# Autodesk Inventor assembly: X-Axis
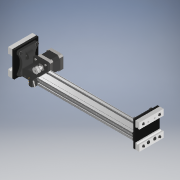
[picture p0: Inventor's stored thumbnail of the model, 180x180]
Saved by Autodesk Inventor 2020.2 (Build 242310000, 310)
## iProperties
Created: 2020-04-02
Part Number: X-Axis
Document SubType Name: Assembly
Designer: rah75
Author: rah75
## Documents named in this file (19)
- C:\Users\rah75\Documents\GitHub\LETU-Maker\CAD\Autodesk Inventor\Base_3001-5999\X-Axis\Assemblies\X-Axis.iam
- C:\Users\rah75\Documents\GitHub\LETU-Maker\CAD\Autodesk Inventor\Base_3001-5999\X-Axis\Fabricated_Parts\X-Axis_Makerslide_LM3003.ipt
- C:\Users\rah75\Documents\GitHub\LETU-Maker\CAD\Autodesk Inventor\Base_3001-5999\X-Axis\Printed_Parts\X-Axis_Carriage_Mount_L_LM3001.ipt
- C:\Users\rah75\Documents\GitHub\LETU-Maker\CAD\Autodesk Inventor\Base_3001-5999\X-Axis\Printed_Parts\X-Axis_Carriage_Mount_R_LM3002.ipt
- C:\Users\rah75\Documents\GitHub\LETU-Maker\CAD\Autodesk Inventor\Base_3001-5999\X-Axis\Fabricated_Parts\X-Axis_End_Plate_LM3004.ipt
- C:\Users\rah75\Documents\GitHub\LETU-Maker\CAD\Autodesk Inventor\Base_3001-5999\X-Axis\Printed_Parts\X-Axis_Mount_Slide_LM3005.ipt
- C:\Users\rah75\Documents\GitHub\LETU-Maker\CAD\Autodesk Inventor\Stock_Components_1001-2999\Motors\NEMA_17_LM1028.ipt
- C:\Users\rah75\Documents\GitHub\LETU-Maker\CAD\Autodesk Inventor\Stock_Components_1001-2999\Power_Transmission\GT2_pulley_LM1034.ipt
- C:\Users\rah75\Documents\GitHub\LETU-Maker\CAD\Autodesk Inventor\Stock_Components_1001-2999\Fasteners\Nuts\hex_nut_m5_LM1020.ipt
- C:\Users\rah75\Documents\GitHub\LETU-Maker\CAD\Autodesk Inventor\Stock_Components_1001-2999\Fasteners\Washers_Spacers\washer_m5_LM1002.ipt
- C:\Users\rah75\Documents\GitHub\LETU-Maker\CAD\Autodesk Inventor\Stock_Components_1001-2999\Fasteners\Screws\BHHD_m5x30_LM1004.ipt
- C:\Users\rah75\Documents\GitHub\LETU-Maker\CAD\Autodesk Inventor\Stock_Components_1001-2999\Fasteners\Screws\SHCS_m3x8_LM1008.ipt
- C:\Users\rah75\Documents\GitHub\LETU-Maker\CAD\Autodesk Inventor\Stock_Components_1001-2999\Fasteners\Screws\SHCS_m3x30_LM1012.ipt
- C:\Users\rah75\Documents\GitHub\LETU-Maker\CAD\Autodesk Inventor\Stock_Components_1001-2999\Power_Transmission\Bearings\623-SS_3x10mm_LM1029.ipt
- C:\Users\rah75\Documents\GitHub\LETU-Maker\CAD\Autodesk Inventor\Stock_Components_1001-2999\Fasteners\Screws\BHHD_m5x45_LM1005.ipt
- C:\Users\rah75\Documents\GitHub\LETU-Maker\CAD\Autodesk Inventor\Stock_Components_1001-2999\Fasteners\Screws\BHHS_m5x80_LM1039.ipt
- C:\Users\rah75\Documents\GitHub\LETU-Maker\CAD\Autodesk Inventor\Stock_Components_1001-2999\Electrical\limit_switch_LM1025.ipt
- C:\Users\rah75\Documents\GitHub\LETU-Maker\CAD\Autodesk Inventor\Stock_Components_1001-2999\Fasteners\Screws\BHHD_m2x10_LM1040.ipt
- C:\Users\rah75\Documents\GitHub\LETU-Maker\CAD\Autodesk Inventor\Stock_Components_1001-2999\Springs\spring_7_5x10mm_LM1036.ipt
## Components (48 placed, 18 different names)
1. X-Axis_Makerslide_LM3003:1 — Insert:1, Mate:1, Insert:2, Mate:2
2. X-Axis_Carriage_Mount_L_LM3001:1 — Insert:2, Mate:2, Insert:4, Mate:4, Insert:8, Mate:10, Insert:25, Insert:26, Insert:28, Insert:29, Insert:30, Insert:31, Insert:32, Insert:40, Mate:11, Insert:43, Mate:14
3. X-Axis_Carriage_Mount_R_LM3002:1 — Insert:1, Mate:1, Insert:3, Mate:3, Mate:7, Insert:18, Insert:20, Insert:22, Insert:27, Insert:33, Insert:35, Mate:12, Mate:13, Angle:1, Mate:16, Mate:17
4. X-Axis_End_Plate_LM3004:1 — Insert:3, Mate:3, Insert:5, Mate:5, Mate:6
5. X-Axis_End_Plate_LM3004:2 — Insert:4, Mate:4, Insert:6, Mate:8, Insert:7, Mate:9
6. X-Axis_Mount_Slide_LM3005:1 — Insert:6, Mate:8, Insert:12, Insert:13, Insert:38, Insert:39
7. X-Axis_Mount_Slide_LM3005:2 — Insert:7, Mate:9, Insert:10, Insert:11
8. X-Axis_Mount_Slide_LM3005:3 — Flush:1, Mate:6, Mate:7, Insert:14, Insert:17
9. X-Axis_Mount_Slide_LM3005:4 — Insert:5, Mate:5, Flush:1, Insert:15, Insert:16, Insert:36, Insert:37
10. NEMA_17_LM1028:1 — Insert:8, Mate:10, Insert:9
11. GT2_pulley_LM1034:1 — Insert:9
12. hex_nut_m5_LM1020:1 — Insert:16
13. hex_nut_m5_LM1020:2 — Insert:12
14. hex_nut_m5_LM1020:3 — Insert:11
15. hex_nut_m5_LM1020:4 — Insert:10
16. hex_nut_m5_LM1020:5 — Insert:15
17. hex_nut_m5_LM1020:6 — Insert:14
18. hex_nut_m5_LM1020:7 — Insert:13
19. hex_nut_m5_LM1020:8 — Insert:17
20. washer_m5_LM1002:1 — Insert:24, Insert:26
21. washer_m5_LM1002:2 — Insert:23, Insert:25
22. washer_m5_LM1002:3 — Insert:19, Insert:20
23. washer_m5_LM1002:4 — Insert:21, Insert:22
24. BHHD_m5x30_LM1004:1 — Insert:23
25. BHHD_m5x30_LM1004:2 — Insert:24
26. BHHD_m5x30_LM1004:3 — Insert:19
27. BHHD_m5x30_LM1004:4 — Insert:21
28. BHHD_m5x30_LM1004:5 — Insert:18
29. BHHD_m5x30_LM1004:6 — Insert:28
30. BHHD_m5x30_LM1004:7 — Insert:27
31. BHHD_m5x30_LM1004:8 — Insert:29
32. SHCS_m3x8_LM1008:1 — Insert:30
33. SHCS_m3x8_LM1008:2 — Insert:31
34. SHCS_m3x8_LM1008:3 — Insert:32
35. SHCS_m3x30_LM1012:1 — Insert:33
36. 623-SS_3x10mm_LM1029:1 — Insert:34
37. 623-SS_3x10mm_LM1029:2 — Insert:34, Insert:35
38. BHHD_m5x45_LM1005:1 — Insert:36
39. BHHD_m5x45_LM1005:2 — Insert:37
40. BHHS_m5x80_LM1039:1 — Insert:38
41. BHHS_m5x80_LM1039:2 — Insert:39
42. limit_switch_LM1025:1 — Insert:40, Mate:11, Insert:41, Insert:42
43. BHHD_m2x10_LM1040:1 — Insert:41
44. BHHD_m2x10_LM1040:2 — Insert:42
45. hex_nut_m5_LM1020:9 — Mate:12, Mate:13, Angle:1
46. hex_nut_m5_LM1020:10 — Insert:43, Mate:15
47. spring_7_5x10mm_LM1036:1 — Mate:14, Mate:15
48. spring_7_5x10mm_LM1036:2 — Mate:16, Mate:17
## Relationships (62: Insert 43, Mate 17, Flush 1, Angle 1)
- Insert:1: X-Axis_Makerslide_LM3003:1 ↔ X-Axis_Carriage_Mount_R_LM3002:1
- Mate:1: X-Axis_Makerslide_LM3003:1 ↔ X-Axis_Carriage_Mount_R_LM3002:1
- Insert:2: X-Axis_Makerslide_LM3003:1 ↔ X-Axis_Carriage_Mount_L_LM3001:1
- Mate:2: X-Axis_Makerslide_LM3003:1 ↔ X-Axis_Carriage_Mount_L_LM3001:1
- Insert:3: X-Axis_Carriage_Mount_R_LM3002:1 ↔ X-Axis_End_Plate_LM3004:1
- Mate:3: X-Axis_Carriage_Mount_R_LM3002:1 ↔ X-Axis_End_Plate_LM3004:1
- Insert:4: X-Axis_Carriage_Mount_L_LM3001:1 ↔ X-Axis_End_Plate_LM3004:2
- Mate:4: X-Axis_Carriage_Mount_L_LM3001:1 ↔ X-Axis_End_Plate_LM3004:2
- Insert:5: X-Axis_End_Plate_LM3004:1 ↔ X-Axis_Mount_Slide_LM3005:4
- Mate:5: X-Axis_End_Plate_LM3004:1 ↔ X-Axis_Mount_Slide_LM3005:4
- Flush:1: X-Axis_Mount_Slide_LM3005:3 ↔ X-Axis_Mount_Slide_LM3005:4
- Mate:6: X-Axis_End_Plate_LM3004:1 ↔ X-Axis_Mount_Slide_LM3005:3
- Mate:7: X-Axis_Carriage_Mount_R_LM3002:1 ↔ X-Axis_Mount_Slide_LM3005:3
- Insert:6: X-Axis_End_Plate_LM3004:2 ↔ X-Axis_Mount_Slide_LM3005:1
- Mate:8: X-Axis_End_Plate_LM3004:2 ↔ X-Axis_Mount_Slide_LM3005:1
- Insert:7: X-Axis_End_Plate_LM3004:2 ↔ X-Axis_Mount_Slide_LM3005:2
- Mate:9: X-Axis_End_Plate_LM3004:2 ↔ X-Axis_Mount_Slide_LM3005:2
- Insert:8: X-Axis_Carriage_Mount_L_LM3001:1 ↔ NEMA_17_LM1028:1
- Mate:10: X-Axis_Carriage_Mount_L_LM3001:1 ↔ NEMA_17_LM1028:1
- Insert:9 (5 mm): NEMA_17_LM1028:1 ↔ GT2_pulley_LM1034:1
- Insert:10: X-Axis_Mount_Slide_LM3005:2 ↔ hex_nut_m5_LM1020:4
- Insert:11: X-Axis_Mount_Slide_LM3005:2 ↔ hex_nut_m5_LM1020:3
- Insert:12: X-Axis_Mount_Slide_LM3005:1 ↔ hex_nut_m5_LM1020:2
- Insert:13: X-Axis_Mount_Slide_LM3005:1 ↔ hex_nut_m5_LM1020:7
- Insert:14: X-Axis_Mount_Slide_LM3005:3 ↔ hex_nut_m5_LM1020:6
- Insert:15: X-Axis_Mount_Slide_LM3005:4 ↔ hex_nut_m5_LM1020:5
- Insert:16: X-Axis_Mount_Slide_LM3005:4 ↔ hex_nut_m5_LM1020:1
- Insert:17: X-Axis_Mount_Slide_LM3005:3 ↔ hex_nut_m5_LM1020:8
- Insert:18: X-Axis_Carriage_Mount_R_LM3002:1 ↔ BHHD_m5x30_LM1004:5
- Insert:19: washer_m5_LM1002:3 ↔ BHHD_m5x30_LM1004:3
- Insert:20: X-Axis_Carriage_Mount_R_LM3002:1 ↔ washer_m5_LM1002:3
- Insert:21: washer_m5_LM1002:4 ↔ BHHD_m5x30_LM1004:4
- Insert:22: X-Axis_Carriage_Mount_R_LM3002:1 ↔ washer_m5_LM1002:4
- Insert:23: washer_m5_LM1002:2 ↔ BHHD_m5x30_LM1004:1
- Insert:24: washer_m5_LM1002:1 ↔ BHHD_m5x30_LM1004:2
- Insert:25: X-Axis_Carriage_Mount_L_LM3001:1 ↔ washer_m5_LM1002:2
- Insert:26: X-Axis_Carriage_Mount_L_LM3001:1 ↔ washer_m5_LM1002:1
- Insert:27: X-Axis_Carriage_Mount_R_LM3002:1 ↔ BHHD_m5x30_LM1004:7
- Insert:28: X-Axis_Carriage_Mount_L_LM3001:1 ↔ BHHD_m5x30_LM1004:6
- Insert:29: X-Axis_Carriage_Mount_L_LM3001:1 ↔ BHHD_m5x30_LM1004:8
- Insert:30: X-Axis_Carriage_Mount_L_LM3001:1 ↔ SHCS_m3x8_LM1008:1
- Insert:31: X-Axis_Carriage_Mount_L_LM3001:1 ↔ SHCS_m3x8_LM1008:2
- Insert:32: X-Axis_Carriage_Mount_L_LM3001:1 ↔ SHCS_m3x8_LM1008:3
- Insert:33: X-Axis_Carriage_Mount_R_LM3002:1 ↔ SHCS_m3x30_LM1012:1
- Insert:34: 623-SS_3x10mm_LM1029:1 ↔ 623-SS_3x10mm_LM1029:2
- Insert:35: X-Axis_Carriage_Mount_R_LM3002:1 ↔ 623-SS_3x10mm_LM1029:2
- Insert:36: X-Axis_Mount_Slide_LM3005:4 ↔ BHHD_m5x45_LM1005:1
- Insert:37: X-Axis_Mount_Slide_LM3005:4 ↔ BHHD_m5x45_LM1005:2
- Insert:38: X-Axis_Mount_Slide_LM3005:1 ↔ BHHS_m5x80_LM1039:1
- Insert:39: X-Axis_Mount_Slide_LM3005:1 ↔ BHHS_m5x80_LM1039:2
- Insert:40: X-Axis_Carriage_Mount_L_LM3001:1 ↔ limit_switch_LM1025:1
- Mate:11: X-Axis_Carriage_Mount_L_LM3001:1 ↔ limit_switch_LM1025:1
- Insert:41: limit_switch_LM1025:1 ↔ BHHD_m2x10_LM1040:1
- Insert:42: limit_switch_LM1025:1 ↔ BHHD_m2x10_LM1040:2
- Mate:12: X-Axis_Carriage_Mount_R_LM3002:1 ↔ hex_nut_m5_LM1020:9
- Mate:13: X-Axis_Carriage_Mount_R_LM3002:1 ↔ hex_nut_m5_LM1020:9
- Angle:1 (0 deg): X-Axis_Carriage_Mount_R_LM3002:1 ↔ hex_nut_m5_LM1020:9
- Insert:43: X-Axis_Carriage_Mount_L_LM3001:1 ↔ hex_nut_m5_LM1020:10
- Mate:14: X-Axis_Carriage_Mount_L_LM3001:1 ↔ spring_7_5x10mm_LM1036:1
- Mate:15: hex_nut_m5_LM1020:10 ↔ spring_7_5x10mm_LM1036:1
- Mate:16: X-Axis_Carriage_Mount_R_LM3002:1 ↔ spring_7_5x10mm_LM1036:2
- Mate:17: X-Axis_Carriage_Mount_R_LM3002:1 ↔ spring_7_5x10mm_LM1036:2
